# Autodesk Inventor assembly: Antena 3 dBi 5.8 GHz v3
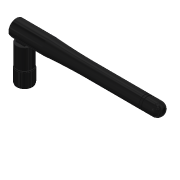
[picture p0: Inventor's stored thumbnail of the model, 180x180]
Saved by Autodesk Inventor 2019 (Build 230136000, 136)
## iProperties
Created: 2020-02-11
Part Number: Antena 3 dBi 5.8 GHz v3
Document SubType Name: Assembly
Designer: Juan Carlos Botero
Author: Juan Carlos Botero
## Documents named in this file (6)
- D:\Drives\OneDrive\Carlos_2\02 TRABAJOS\MULTIPLO\Antena 3 dBi 5.8 GHz v3.iam
- D:\Drives\OneDrive\Carlos_2\02 TRABAJOS\MULTIPLO\Conveyor\ENSAMBLE - Copy\Solid1_1.ipt
- D:\Drives\OneDrive\Carlos_2\02 TRABAJOS\MULTIPLO\Conveyor\ENSAMBLE - Copy\Solid2_1.ipt
- D:\Drives\OneDrive\Carlos_2\02 TRABAJOS\MULTIPLO\Conveyor\ENSAMBLE - Copy\Solid3.ipt
- D:\Drives\OneDrive\Carlos_2\02 TRABAJOS\MULTIPLO\Conveyor\ENSAMBLE - Copy\Solid4.ipt
- D:\Drives\OneDrive\Carlos_2\02 TRABAJOS\MULTIPLO\Conveyor\ENSAMBLE - Copy\Solid5.ipt
## Components (5 placed, 5 different names)
1. Solid1_1:1
2. Solid2_1:1 — Rotational:1
3. Solid3:1
4. Solid4:1
5. Solid5:1 — Rotational:1
## Relationships (1: RevoluteJoint 1)
- Rotational:1 [RevoluteJoint]: Solid2_1:1 ↔ Solid5:1
